# Autodesk Inventor assembly: CameraSetup
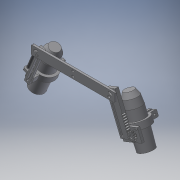
[picture p0: Inventor's stored thumbnail of the model, 180x180]
Saved by Autodesk Inventor 2019 (Build 230136000, 136)
## iProperties
Created: 2019-07-15
Part Number: CameraSetup
Document SubType Name: Assembly
Designer: aorfi
Author: aorfi
## Documents named in this file (11)
- C:\Users\aorfi\Documents\IQC\CameraSetup.iam
- C:\Users\aorfi\Documents\IQC\COTS\USBCamera.ipt
- C:\Users\aorfi\Documents\IQC\CustomParts\CameraClamp.ipt
- C:\Users\aorfi\Documents\IQC\CustomParts\CameraSlider.ipt
- C:\Users\aorfi\Documents\IQC\CustomParts\CameraBase.ipt
- C:\Users\aorfi\Documents\IQC\CustomParts\StopRotation.ipt
- C:\Users\aorfi\Documents\IQC\CustomParts\LeadScrew.ipt
- C:\Users\aorfi\Documents\IQC\CustomParts\Rack.ipt
- C:\Users\aorfi\Documents\IQC\CustomParts\Pinion.ipt
- C:\Users\aorfi\Documents\IQC\CustomParts\PinionHolder.ipt
- C:\Users\aorfi\Documents\IQC\CustomParts\Pawl.ipt
## Components (12 placed, 10 different names)
1. USBCamera:2 — Mate:2, Symmetry:1, Mate:10
2. CameraClamp:1 — Mate:1, Angle:1, Symmetry:2, Mate:11, Tangent:1, Mate:15, Mate:16, Mate:17
3. USBCamera:1 — Mate:1, Symmetry:1, Mate:11
4. CameraClamp:2 — Mate:2, Symmetry:2, Mate:10, Mate:24, Mate:25, Flush:3
5. CameraSlider:1 — Angle:1, Mate:8, Tangent:1, Mate:18, Mate:19, Symmetry:3
6. CameraBase:1 — Flush:1, Mate:8, Mate:12, Mate:14, Mate:19, Mate:21
7. StopRotation:1 — Mate:15, Mate:16, Mate:17, Mate:18, Mate:20
8. LeadScrew:1 — Mate:20
9. Rack:1 — Mate:21, Symmetry:3, Mate:27, Mate:28
10. Pinion:1 — Mate:29, Mate:30
11. PinionHolder:1 — Mate:24, Mate:25, Flush:3, Mate:27, Mate:28, Mate:29, Mate:30, Mate:31, Mate:32
12. Pawl:1 — Mate:31, Mate:32
## Relationships (29: Mate 22, Symmetry 3, Flush 2, Angle 1, Tangent 1)
- Mate:1: CameraClamp:1 ↔ USBCamera:1
- Mate:2: USBCamera:2 ↔ CameraClamp:2
- Angle:1 (0 deg): CameraClamp:1 ↔ CameraSlider:1
- Flush:1: CameraBase:1
- Mate:8: CameraSlider:1 ↔ CameraBase:1
- Symmetry:1: USBCamera:2 ↔ USBCamera:1
- Symmetry:2: CameraClamp:1 ↔ CameraClamp:2
- Mate:10: USBCamera:2 ↔ CameraClamp:2
- Mate:11: CameraClamp:1 ↔ USBCamera:1
- Mate:12: CameraBase:1
- Mate:14: CameraBase:1
- Tangent:1: CameraClamp:1 ↔ CameraSlider:1
- Mate:15: CameraClamp:1 ↔ StopRotation:1
- Mate:16: CameraClamp:1 ↔ StopRotation:1
- Mate:17: CameraClamp:1 ↔ StopRotation:1
- Mate:18: CameraSlider:1 ↔ StopRotation:1
- Mate:19: CameraSlider:1 ↔ CameraBase:1
- Mate:20: StopRotation:1 ↔ LeadScrew:1
- Mate:21: CameraBase:1 ↔ Rack:1
- Symmetry:3: CameraSlider:1 ↔ Rack:1
- Mate:24: CameraClamp:2 ↔ PinionHolder:1
- Mate:25: CameraClamp:2 ↔ PinionHolder:1
- Flush:3: CameraClamp:2 ↔ PinionHolder:1
- Mate:27: Rack:1 ↔ PinionHolder:1
- Mate:28: Rack:1 ↔ PinionHolder:1
- Mate:29: Pinion:1 ↔ PinionHolder:1
- Mate:30: Pinion:1 ↔ PinionHolder:1
- Mate:31: PinionHolder:1 ↔ Pawl:1
- Mate:32: PinionHolder:1 ↔ Pawl:1
